# Autodesk Inventor assembly: leg_press_assembly
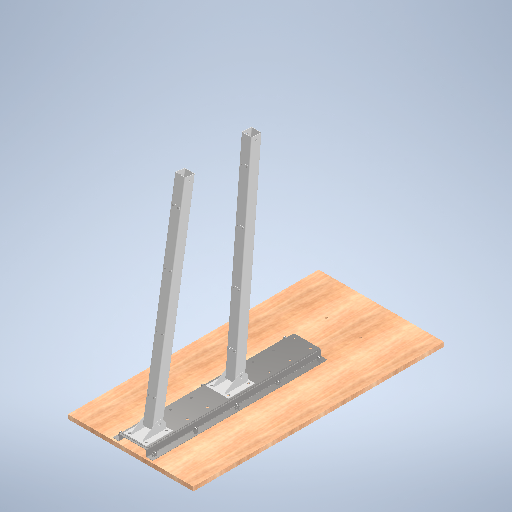
[picture p0: Inventor's stored thumbnail of the model, 512x512]
Saved by Autodesk Inventor 2025.2 (Build 292293000, 293)
## iProperties
Created: 2025-03-24
Part Number: leg_press_assembly
Document SubType Name: Assembly
Designer: Caspe
Author: Caspe
## Documents named in this file (5)
- C:\Users\Caspe\Documents\Semester 8\Project\Anomaly_Detection\Mechanical_Project\Inventor_project\leg_press_assembly.iam
- C:\Users\Caspe\Documents\Semester 8\Project\Anomaly_Detection\Mechanical_Project\Inventor_project\IMS-00-100.iam
- C:\Users\Caspe\Documents\Semester 8\Project\Anomaly_Detection\Mechanical_Project\Inventor_project\bottom_hinge.iam
- C:\Users\Caspe\Documents\Semester 8\Project\Anomaly_Detection\Mechanical_Project\Inventor_project\A1.iam
- C:\Users\Caspe\Documents\Semester 8\Project\Anomaly_Detection\Mechanical_Project\Leg_press_parameters.xlsx
## Components (5 placed, 3 different names)
1. IMS-00-100:1 [sub-assembly] — Insert:1, Insert:2, Insert:3, Insert:4
2. bottom_hinge:1 [sub-assembly] — Insert:1, Insert:2, Mate:1, Mate:2
3. A1:1 [sub-assembly] — Mate:1, Mate:2
4. bottom_hinge:2 [sub-assembly] — Insert:3, Insert:4, Mate:3, Mate:4
5. A1:2 [sub-assembly] — Mate:3, Mate:4
## Relationships (8: Insert 4, Mate 4)
- Insert:1: IMS-00-100:1 ↔ bottom_hinge:1
- Insert:2: IMS-00-100:1 ↔ bottom_hinge:1
- Mate:1: bottom_hinge:1 ↔ A1:1
- Mate:2 (3 mm): bottom_hinge:1 ↔ A1:1
- Insert:3: IMS-00-100:1 ↔ bottom_hinge:2
- Insert:4: IMS-00-100:1 ↔ bottom_hinge:2
- Mate:3: bottom_hinge:2 ↔ A1:2
- Mate:4 (3 mm): bottom_hinge:2 ↔ A1:2
## Named parameters: A_length = 1000 mm, A_width = 50 mm, A_bend = 20 mm, A_connection_width = 40 mm, A_displacement = 500 mm, A_hole_height = 10 mm, A_hole_length = 40 mm, A_joint_diameter = 10 mm, A_height = 50 mm, A_joint_tolerance = 3 mm, l___________ = 0 mm, B_length = 1200 mm, B_width = 50 mm, B_bend = 20 mm, B_connection_width = 40 mm, B_hole_height = 10 mm, B_hole_length = 40 mm, l__________ = 0 mm, C_length = 300 mm, C_width = 20 mm, C_height = 400 mm, l_________ = 0 mm, rivet_diameter = 4 mm, rivet_displacement = 250 mm, plate_thickness = 2 mm, l________ = 0 mm
